# Autodesk Inventor assembly: Water Table 4x4
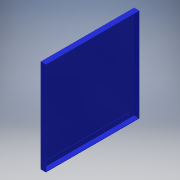
[picture p0: Inventor's stored thumbnail of the model, 180x180]
Saved by Autodesk Inventor 2018.2 (Build 222227000, 227)
## iProperties
Created: 2017-12-19
Part Number: Water Table 4x4
Document SubType Name: Assembly
Designer: torba
Author: torba
## Documents named in this file (5)
- C:\Users\torba\OneDrive\Documents\Inventor\Plasma 5x10\Water Table 4x4.iam
- C:\Users\torba\OneDrive\Documents\Inventor\Plasma 5x10\3 x 3 angle 45 .25 steel.ipt
- C:\Users\torba\OneDrive\Documents\Inventor\Plasma 5x10\1-16 sheet metal.ipt
- C:\Users\torba\OneDrive\Documents\Inventor\Plasma 5x10\1-16 sheet metal\1-16 sheet metal-48x48.ipt
- C:\Users\torba\OneDrive\Documents\Inventor\Plasma 5x10\3 x 3 angle 45 .25 steel\3 x 3 angle 45 .25 steel-54.ipt
## Components (5 placed, 2 different names)
1. 3 x 3 angle 45 .25 steel-54:1 — Flush:2, Mate:3, Mate:4, Flush:3, Mate:6
2. 3 x 3 angle 45 .25 steel-54:2 — Mate:1, Flush:1, Mate:2, Mate:5, Flush:4, Mate:10
3. 3 x 3 angle 45 .25 steel-54:3 — Mate:1, Flush:1, Mate:2, Flush:2, Mate:3, Mate:4
4. 3 x 3 angle 45 .25 steel-54:4 — Flush:3, Mate:5, Mate:6, Mate:11
5. 1-16 sheet metal-48x48:1 — Flush:4, Mate:10, Mate:11
## Relationships (12: Mate 8, Flush 4)
- Mate:1: 3 x 3 angle 45 .25 steel-54:2 ↔ 3 x 3 angle 45 .25 steel-54:3
- Flush:1: 3 x 3 angle 45 .25 steel-54:2 ↔ 3 x 3 angle 45 .25 steel-54:3
- Mate:2: 3 x 3 angle 45 .25 steel-54:2 ↔ 3 x 3 angle 45 .25 steel-54:3
- Flush:2: 3 x 3 angle 45 .25 steel-54:1 ↔ 3 x 3 angle 45 .25 steel-54:3
- Mate:3: 3 x 3 angle 45 .25 steel-54:1 ↔ 3 x 3 angle 45 .25 steel-54:3
- Mate:4: 3 x 3 angle 45 .25 steel-54:1 ↔ 3 x 3 angle 45 .25 steel-54:3
- Flush:3: 3 x 3 angle 45 .25 steel-54:1 ↔ 3 x 3 angle 45 .25 steel-54:4
- Mate:5: 3 x 3 angle 45 .25 steel-54:2 ↔ 3 x 3 angle 45 .25 steel-54:4
- Mate:6: 3 x 3 angle 45 .25 steel-54:1 ↔ 3 x 3 angle 45 .25 steel-54:4
- Flush:4: 3 x 3 angle 45 .25 steel-54:2 ↔ 1-16 sheet metal-48x48:1
- Mate:10: 3 x 3 angle 45 .25 steel-54:2 ↔ 1-16 sheet metal-48x48:1
- Mate:11: 3 x 3 angle 45 .25 steel-54:4 ↔ 1-16 sheet metal-48x48:1
